# Autodesk Inventor assembly: 50-J5
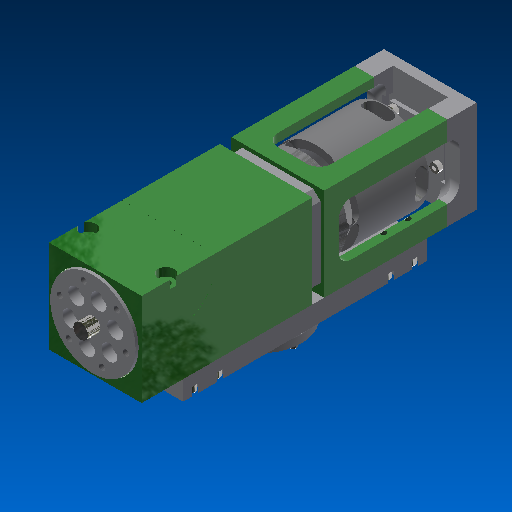
[picture p0: Inventor's stored thumbnail of the model, 512x512]
Saved by Autodesk Inventor 2018 (Build 220112000, 112)
## iProperties
Created: 2020-07-02
Part Number: 50-J5
Document SubType Name: Assembly
Designer: Bunny320
Author: Bunny320
## Documents named in this file (13)
- C:\Users\Bunny320\Desktop\sechs\4-CAD\50-J5.iam
- C:\Users\Bunny320\Desktop\sechs\4-CAD\motor unit 2820.iam
- C:\Users\Bunny320\Desktop\sechs\4-CAD\502-gearbox-housing.ipt
- C:\Users\Bunny320\Desktop\sechs\4-CAD\standardParts\61705-2RZ\W 61705-2RZ.iam
- C:\Users\Bunny320\Desktop\sechs\4-CAD\504-shaft.ipt
- C:\Users\Bunny320\Desktop\sechs\4-CAD\403-coupler dummy.ipt
- C:\Users\Bunny320\Desktop\sechs\4-CAD\standardParts\Pololu mounting hub\pololu-universal-aluminum-mounting-hub-for-6mm-shaft-m3-holes.ipt
- C:\Users\Bunny320\Desktop\sechs\4-CAD\501-flange.ipt
- C:\Users\Bunny320\Desktop\sechs\4-CAD\502-gearbox-housing-cap.ipt
- C:\Users\Bunny320\Documents\Inventor\Content Center Files\R2018\en-US\ISO 10642(2)\ISO 10642  - M3  x  12.ipt
- C:\Users\Bunny320\Documents\Inventor\Content Center Files\R2018\en-US\ISO 4762(1)\DIN EN ISO 4762 - M3 x 12.ipt
- C:\Users\Bunny320\Documents\Inventor\Content Center Files\R2018\en-US\ISO 4762(1)\DIN EN ISO 4762 - M3 x 8.ipt
- C:\Users\Bunny320\Desktop\sechs\4-CAD\505-output disk.ipt
## Components (27 placed, 12 different names)
1. motor unit 2820:1 [sub-assembly] — Flush:1, Flush:2, Flush:3, Mate:1, Mate:2, Mate:3, Mate:9, Mate:67, Mate:69, Mate:70
2. 502-gearbox-housing:1 — Mate:1, Mate:2, Mate:3, Mate:6, Mate:15, Mate:16, Mate:17, Mate:18, Mate:19, Mate:20, Mate:21, Mate:22, Mate:74, Mate:76, Mate:77
3. W 61705-2RZ:1 [sub-assembly] — Mate:6, Mate:71, Mate:73, Mate:74, Mate:75
4. 504-shaft:1 — Mate:9
5. pololu-universal-aluminum-mounting-hub-for-6mm-shaft-m3-holes:1 — Mate:72, Mate:73
6. 501-flange:1 — Mate:15, Mate:27, Mate:28, Mate:29, Mate:30, Mate:31, Mate:32, Mate:33, Mate:34, Mate:35, Mate:36, Mate:37, Mate:38, Mate:39, Mate:40, Mate:41, Mate:42, Mate:43, Mate:44, Mate:45, Mate:46, Mate:47, Mate:48, Mate:49, Mate:50, Mate:51, Mate:52, Mate:53, Mate:54, Mate:69, Mate:70
7. 502-gearbox-housing-cap:1 — Mate:16, Mate:17, Mate:18, Mate:76, Mate:77
8. 403-coupler dummy:1 — Mate:67
9. 505-output disk:1 — Mate:71, Mate:72, Mate:75
10. DIN EN ISO 10642 M3  x  12:1 — Mate:19
11. DIN EN ISO 10642 M3  x  12:2 — Mate:20
12. DIN EN ISO 10642 M3  x  12:3 — Mate:21
13. DIN EN ISO 10642 M3  x  12:4 — Mate:22
14. DIN EN ISO 4762 M3 x 12:1 — Mate:27, Mate:28
15. DIN EN ISO 4762 M3 x 12:2 — Mate:29, Mate:30
16. DIN EN ISO 4762 M3 x 12:3 — Mate:31, Mate:32
17. DIN EN ISO 4762 M3 x 12:4 — Mate:33, Mate:34
18. DIN EN ISO 4762 M3 x 12:5 — Mate:35, Mate:36
19. DIN EN ISO 4762 M3 x 12:6 — Mate:37, Mate:38
20. DIN EN ISO 4762 M3 x 8:1 — Mate:39, Mate:40
21. DIN EN ISO 4762 M3 x 8:2 — Mate:41, Mate:42
22. DIN EN ISO 4762 M3 x 8:3 — Mate:43, Mate:44
23. DIN EN ISO 4762 M3 x 8:4 — Mate:45, Mate:46
24. DIN EN ISO 4762 M3 x 8:5 — Mate:47, Mate:48
25. DIN EN ISO 4762 M3 x 8:6 — Mate:49, Mate:50
26. DIN EN ISO 4762 M3 x 8:7 — Mate:51, Mate:52
27. DIN EN ISO 4762 M3 x 8:8 — Mate:53, Mate:54
## Relationships (54: Mate 51, Flush 3)
- Flush:1: motor unit 2820:1
- Flush:2: motor unit 2820:1
- Flush:3: motor unit 2820:1
- Mate:1: motor unit 2820:1 ↔ 502-gearbox-housing:1
- Mate:2: motor unit 2820:1 ↔ 502-gearbox-housing:1
- Mate:3: motor unit 2820:1 ↔ 502-gearbox-housing:1
- Mate:6: 502-gearbox-housing:1 ↔ W 61705-2RZ:1
- Mate:9: motor unit 2820:1 ↔ 504-shaft:1
- Mate:15: 502-gearbox-housing:1 ↔ 501-flange:1
- Mate:16: 502-gearbox-housing:1 ↔ 502-gearbox-housing-cap:1
- Mate:17: 502-gearbox-housing:1 ↔ 502-gearbox-housing-cap:1
- Mate:18: 502-gearbox-housing:1 ↔ 502-gearbox-housing-cap:1
- Mate:19: 502-gearbox-housing:1 ↔ DIN EN ISO 10642 M3  x  12:1
- Mate:20: 502-gearbox-housing:1 ↔ DIN EN ISO 10642 M3  x  12:2
- Mate:21: 502-gearbox-housing:1 ↔ DIN EN ISO 10642 M3  x  12:3
- Mate:22: 502-gearbox-housing:1 ↔ DIN EN ISO 10642 M3  x  12:4
- Mate:27: 501-flange:1 ↔ DIN EN ISO 4762 M3 x 12:1
- Mate:28: 501-flange:1 ↔ DIN EN ISO 4762 M3 x 12:1
- Mate:29: 501-flange:1 ↔ DIN EN ISO 4762 M3 x 12:2
- Mate:30: 501-flange:1 ↔ DIN EN ISO 4762 M3 x 12:2
- Mate:31: 501-flange:1 ↔ DIN EN ISO 4762 M3 x 12:3
- Mate:32: 501-flange:1 ↔ DIN EN ISO 4762 M3 x 12:3
- Mate:33: 501-flange:1 ↔ DIN EN ISO 4762 M3 x 12:4
- Mate:34: 501-flange:1 ↔ DIN EN ISO 4762 M3 x 12:4
- Mate:35: 501-flange:1 ↔ DIN EN ISO 4762 M3 x 12:5
- Mate:36: 501-flange:1 ↔ DIN EN ISO 4762 M3 x 12:5
- Mate:37: 501-flange:1 ↔ DIN EN ISO 4762 M3 x 12:6
- Mate:38: 501-flange:1 ↔ DIN EN ISO 4762 M3 x 12:6
- Mate:39: 501-flange:1 ↔ DIN EN ISO 4762 M3 x 8:1
- Mate:40: 501-flange:1 ↔ DIN EN ISO 4762 M3 x 8:1
- Mate:41: 501-flange:1 ↔ DIN EN ISO 4762 M3 x 8:2
- Mate:42: 501-flange:1 ↔ DIN EN ISO 4762 M3 x 8:2
- Mate:43: 501-flange:1 ↔ DIN EN ISO 4762 M3 x 8:3
- Mate:44: 501-flange:1 ↔ DIN EN ISO 4762 M3 x 8:3
- Mate:45: 501-flange:1 ↔ DIN EN ISO 4762 M3 x 8:4
- Mate:46: 501-flange:1 ↔ DIN EN ISO 4762 M3 x 8:4
- Mate:47: 501-flange:1 ↔ DIN EN ISO 4762 M3 x 8:5
- Mate:48: 501-flange:1 ↔ DIN EN ISO 4762 M3 x 8:5
- Mate:49: 501-flange:1 ↔ DIN EN ISO 4762 M3 x 8:6
- Mate:50: 501-flange:1 ↔ DIN EN ISO 4762 M3 x 8:6
- Mate:51: 501-flange:1 ↔ DIN EN ISO 4762 M3 x 8:7
- Mate:52: 501-flange:1 ↔ DIN EN ISO 4762 M3 x 8:7
- Mate:53: 501-flange:1 ↔ DIN EN ISO 4762 M3 x 8:8
- Mate:54: 501-flange:1 ↔ DIN EN ISO 4762 M3 x 8:8
- Mate:67: motor unit 2820:1 ↔ 403-coupler dummy:1
- Mate:69: motor unit 2820:1 ↔ 501-flange:1
- Mate:70: motor unit 2820:1 ↔ 501-flange:1
- Mate:71: W 61705-2RZ:1 ↔ 505-output disk:1
- Mate:72: pololu-universal-aluminum-mounting-hub-for-6mm-shaft-m3-holes:1 ↔ 505-output disk:1
- Mate:73: W 61705-2RZ:1 ↔ pololu-universal-aluminum-mounting-hub-for-6mm-shaft-m3-holes:1
- Mate:74: 502-gearbox-housing:1 ↔ W 61705-2RZ:1
- Mate:75: W 61705-2RZ:1 ↔ 505-output disk:1
- Mate:76: 502-gearbox-housing:1 ↔ 502-gearbox-housing-cap:1
- Mate:77: 502-gearbox-housing:1 ↔ 502-gearbox-housing-cap:1
